# Autodesk Inventor assembly: ASY MSC 002 отстойник осветлитель
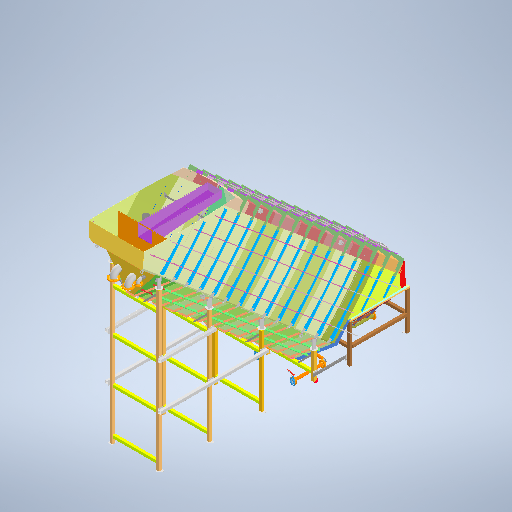
[picture p0: Inventor's stored thumbnail of the model, 512x512]
Saved by Autodesk Inventor 2025 (Build 290162010, 162A)
## iProperties
allow_slope_adjustment: 0 ul
flow_configuration: 1 ul
flow_direction: 2 ul
loss_method: 0 ul
radius: 110.000 mm
flow_configuration2: 1 ul
radius: 61.000 mm
radius: 44.450 mm
radius: 59.000 mm
Created: 2024-09-05
Part Number: ASY MSC 002 отстойник осветлитель
Document SubType Name: Assembly
Designer: admin
Mass: 3.32015e+06 g
Surface Area: 6.08051e+06 cm^2
Volume: 432456 cm^3
Author: admin
## Documents named in this file (64)
- C:\Users\pokla\Documents\Inventor\Отстойник осветлитель\Manturovo_Se-clar-Gleb\ASY MSC 002 отстойник осветлитель.iam
- C:\Users\pokla\Documents\Inventor\Отстойник осветлитель\Manturovo_Se-clar-Gleb\ASY MSC 900.1 base frame.iam
- C:\Users\pokla\Documents\Inventor\Отстойник осветлитель\Manturovo_Se-clar-Gleb\ASY MSC 100 cone.iam
- C:\Users\pokla\Documents\Inventor\Отстойник осветлитель\Manturovo_Se-clar-Gleb\MSC 401 sheet lowerback.ipt
- C:\Users\pokla\Documents\Inventor\Отстойник осветлитель\Manturovo_Se-clar-Gleb\MSC 701 face 1.ipt
- C:\Users\pokla\Documents\Inventor\Отстойник осветлитель\Manturovo_Se-clar-Gleb\MSC 705 ridge 3.ipt
- C:\Users\pokla\Documents\Inventor\Отстойник осветлитель\Manturovo_Se-clar-Gleb\MSC 713 tube.ipt
- C:\Users\pokla\Documents\Inventor\Отстойник осветлитель\Manturovo_Se-clar-Gleb\ISO 5251 Bends 3D without straight ends(90 deg) DN150 11 11.ipt
- C:\Users\pokla\Documents\Inventor\Отстойник осветлитель\Manturovo_Se-clar-Gleb\MSC 408 stringer lowerback.ipt
- C:\Users\pokla\Documents\Inventor\Отстойник осветлитель\Manturovo_Se-clar-Gleb\MSC 703 face 2.ipt
- C:\Users\pokla\Documents\Inventor\Отстойник осветлитель\Manturovo_Se-clar-Gleb\MSC 702 face 3.ipt
- C:\Users\pokla\Documents\Inventor\Отстойник осветлитель\Manturovo_Se-clar-Gleb\MSC 704 face 4.ipt
- C:\Users\pokla\Documents\Inventor\Отстойник осветлитель\Manturovo_Se-clar-Gleb\ASY MSC 900.3 base frame.iam
- C:\Users\pokla\Documents\Inventor\Отстойник осветлитель\Manturovo_Se-clar-Gleb\Pillars\ASY MSC 900.5 base frame.iam
- C:\Users\pokla\Documents\Inventor\Отстойник осветлитель\Manturovo_Se-clar-Gleb\Pillars\ASY MSC 900.4  base frame.iam
- C:\Users\pokla\Documents\Inventor\Отстойник осветлитель\Manturovo_Se-clar-Gleb\Pillars\ASY MSC 900.6 base frame.iam
- C:\Users\pokla\Documents\Inventor\Отстойник осветлитель\Manturovo_Se-clar-Gleb\ASY MSC 200 BACK.iam
- C:\Users\pokla\Documents\Inventor\Отстойник осветлитель\Manturovo_Se-clar-Gleb\ASY MSC 300.2 LEFT BOARD.iam
- C:\Users\pokla\Documents\Inventor\Отстойник осветлитель\Manturovo_Se-clar-Gleb\ASY MSC 300.1 RIGHT BOARD.iam
- C:\Users\pokla\Documents\Inventor\Отстойник осветлитель\Manturovo_Se-clar-Gleb\ASY MSC 500 BELLY.iam
- C:\Users\pokla\Documents\Inventor\Отстойник осветлитель\Manturovo_Se-clar-Gleb\ASY MSC 900.2 support.iam
- C:\Users\pokla\Documents\Inventor\Отстойник осветлитель\Manturovo_Se-clar-Gleb\ASY MSC 600 cone exit back.iam
- C:\Users\pokla\Documents\Inventor\Отстойник осветлитель\Manturovo_Se-clar-Gleb\ASY MSC 800 gills.iam
- C:\Users\pokla\Documents\Inventor\Отстойник осветлитель\Manturovo_Se-clar-Gleb\ASY MSC 400 Accsess hatch.iam
- C:\Users\pokla\Documents\Inventor\Отстойник осветлитель\Manturovo_Se-clar-Gleb\MSC DIM 000 settler-clarifier.ipt
- C:\Users\pokla\Documents\Inventor\Отстойник осветлитель\Manturovo_Se-clar-Gleb\MSC DIM 001 frame.ipt
- C:\Users\pokla\Documents\Inventor\Отстойник осветлитель\Manturovo_Se-clar-Gleb\ASY MSC 900.7 base frame transverse.iam
- C:\Users\pokla\Documents\Inventor\Отстойник осветлитель\Manturovo_Se-clar-Gleb\ASY MSC 900.8 base frame transverse.iam
- C:\Users\pokla\Documents\Inventor\Отстойник осветлитель\Manturovo_Se-clar-Gleb\MSC 908 transverse pillar plate.ipt
- C:\Users\pokla\Documents\Inventor\Отстойник осветлитель\Manturovo_Se-clar-Gleb\MSC 900.9 base frame transverse.ipt
- C:\Users\pokla\Documents\Inventor\Отстойник осветлитель\Manturovo_Se-clar-Gleb\ASY MSC 700 water tray.iam
- C:\Users\pokla\Documents\Inventor\Отстойник осветлитель\Manturovo_Se-clar-Gleb\ASY 940 linkage.iam
- C:\Users\pokla\Documents\Inventor\Отстойник осветлитель\Manturovo_Se-clar-Gleb\MSC 510 BELLY PILLAR.ipt
- C:\Users\pokla\Documents\Inventor\Отстойник осветлитель\Manturovo_Se-clar-Gleb\ASY MSC 900.7 support.iam
- C:\Users\pokla\Documents\Inventor\Отстойник осветлитель\Manturovo_Se-clar-Gleb\Content Center Files\en-US\DIN 2605 90 T 3\DIN 2605 90 Deg Elbow Type 2 168.3 - 2.6S.ipt
- C:\Users\admin\YandexDisk-badmisterfox\домашниий пк\Inventor\Manturovo\Manturovo_Se-clar\3d party\Stamp flange DIN2642\Stamd flange lapped collar DIN2642.ipt
- C:\Users\pokla\Documents\Inventor\Отстойник осветлитель\Manturovo_Se-clar-Gleb\3d party\Stamp flange DIN2642\Stamd flange lapped collar DIN2642\Stamp flange DIN2642-150.ipt
- C:\Users\pokla\Documents\Inventor\Отстойник осветлитель\Manturovo_Se-clar-Gleb\Content Center Files\en-US\DIN 2605 90 T 3\DIN 2605 90 Deg Elbow Type 2 88.9 - 2.3S.ipt
- C:\Users\pokla\Documents\Inventor\Отстойник осветлитель\Manturovo_Se-clar-Gleb\Stamp flange DIN2642-080.ipt
- C:\Users\pokla\Documents\Inventor\Отстойник осветлитель\Manturovo_Se-clar-Gleb\DIN EN ISO 1127(1) - 88,9 x 2,3 - 100.ipt
- C:\Users\pokla\Documents\Inventor\Отстойник осветлитель\Manturovo_Se-clar-Gleb\3d party\Butterfly value\butterfly-valve-3-in-1.snapshot.4\vpe_3449-02_dn80_.iam
- C:\Users\pokla\Documents\Inventor\Отстойник осветлитель\Manturovo_Se-clar-Gleb\MSC 606 rocket tube 6.ipt
- C:\Users\pokla\Documents\Inventor\Отстойник осветлитель\Manturovo_Se-clar-Gleb\Stamp flange DIN2642-065.ipt
- C:\Users\pokla\Documents\Inventor\Отстойник осветлитель\Manturovo_Se-clar-Gleb\ContentCenter\en-US\ISO 5251 B 3D\ISO 5251 Bends 3D without straight ends(90 deg) DN65 2.9 2.9.ipt
- C:\Users\pokla\Documents\Inventor\Отстойник осветлитель\Manturovo_Se-clar-Gleb\MSC 616 belly tube 16.ipt
- C:\Users\pokla\Documents\Inventor\Отстойник осветлитель\Manturovo_Se-clar-Gleb\MSC 617 belly tube 17.ipt
- C:\Users\pokla\Documents\Inventor\Отстойник осветлитель\Manturovo_Se-clar-Gleb\MSC 618 belly tube 18.ipt
- C:\Users\pokla\Documents\Inventor\Отстойник осветлитель\Manturovo_Se-clar-Gleb\MSC 808 sheet.ipt
- C:\Users\pokla\Documents\Inventor\Отстойник осветлитель\Manturovo_Se-clar-Gleb\DIN EN 10219-2 - 40 x 20 x 2  - 2000.ipt
- C:\Users\pokla\Documents\Inventor\Отстойник осветлитель\Manturovo_Se-clar-Gleb\ISO 4019 - 40x20x2 - 1600.ipt
- C:\Users\pokla\Documents\Inventor\Отстойник осветлитель\Manturovo_Se-clar-Gleb\MSC 814 wall inner rib.ipt
- C:\Users\pokla\Documents\Inventor\Отстойник осветлитель\Manturovo_Se-clar-Gleb\MSC 815 wall inner.ipt
- C:\Users\pokla\Documents\Inventor\Отстойник осветлитель\Manturovo_Se-clar-Gleb\MSC 815 wall inner joint.ipt
- C:\Users\pokla\Documents\Inventor\Отстойник осветлитель\Manturovo_Se-clar-Gleb\UNI EN ISO 1127(1) - 168.3 x 2 - 700.ipt
- C:\Users\pokla\Documents\Inventor\Отстойник осветлитель\Manturovo_Se-clar-Gleb\MSC 912 flange slipway.ipt
- C:\Users\pokla\Documents\Inventor\Отстойник осветлитель\Manturovo_Se-clar-Gleb\MSC 913 flange slipway.ipt
- C:\Users\pokla\Documents\Inventor\Отстойник осветлитель\Manturovo_Se-clar-Gleb\MSC 920 plug 88.9.ipt
- C:\Users\pokla\Documents\Inventor\Отстойник осветлитель\Manturovo_Se-clar-Gleb\MSC 921 plug 76.ipt
- C:\Users\pokla\Documents\Inventor\Отстойник осветлитель\Manturovo_Se-clar-Gleb\MSC 922 plug 76 hole.ipt
- C:\Users\pokla\Documents\Inventor\Отстойник осветлитель\Manturovo_Se-clar-Gleb\MSC 922 plug 150.ipt
- C:\Users\pokla\Documents\Inventor\Отстойник осветлитель\Manturovo_Se-clar-Gleb\AQUA AISI304 4vv wheel plate 150.ipt
- C:\Users\pokla\Documents\Inventor\Отстойник осветлитель\Manturovo_Se-clar-Gleb\MSC 923 step .ipt
- C:\Users\pokla\Documents\Inventor\Отстойник осветлитель\Manturovo_Se-clar-Gleb\ASY MSC D-ring.iam
- C:\Users\pokla\Documents\Inventor\Отстойник осветлитель\Manturovo_Se-clar-Gleb\3d party\Stamp flange DIN2642\Stamd flange lapped collar DIN2642.ipt
## Components (104 placed, 62 different names)
1. MSC DIM 000 settler-clarifier.ipt:1
2. MSC DIM 001 frame.ipt:1
3. ASY MSC 900.4  base frame.iam:1 [sub-assembly] — Mate:32, Mate:33, Mate:45, Mate:46, Cylindrical:11, Mate:82, Rigid:67
4. ASY MSC 900.5 base frame.iam:1 [sub-assembly] — Flush:11, Cylindrical:7, Mate:46, Mate:48, Cylindrical:10
5. ASY MSC 900.6 base frame.iam:1 [sub-assembly] — Mate:38, Mate:39, Cylindrical:6, Mate:47, Rigid:19, Rigid:20, Rigid:21, Rigid:22, Cylindrical:9, Mate:84
6. ASY MSC 900.3 base frame.iam:1 [sub-assembly] — Mate:23, Mate:24, Mate:44, Mate:45, Rigid:31, Rigid:32, Rigid:33, Cylindrical:8
7. ASY MSC 900.8 base frame transverse.iam:1 [sub-assembly] — Rigid:22
8. ASY MSC 900.8 base frame transverse.iam:2 [sub-assembly] — Rigid:21
9. ASY MSC 900.7 base frame transverse.iam:1 [sub-assembly] — Rigid:19
10. ASY MSC 900.7 base frame transverse.iam:2 [sub-assembly] — Rigid:20
11. ASY MSC 900.2 support.iam:5 [sub-assembly]
12. ASY MSC 900.7 support:2 [sub-assembly] — Cylindrical:11, Mate:78
13. ASY MSC 900.2 support.iam:4 [sub-assembly] — Cylindrical:7, Mate:41
14. ASY MSC 900.7 support:3 [sub-assembly] — Cylindrical:10, Mate:79
15. ASY MSC 900.2 support.iam:1 [sub-assembly] — Cylindrical:6, Mate:42
16. ASY MSC 900.7 support:4 [sub-assembly] — Cylindrical:9, Mate:80
17. ASY MSC 900.2 support.iam:8 [sub-assembly]
18. ASY MSC 900.7 support:1 [sub-assembly] — Cylindrical:8, Mate:77
19. ASY MSC 600 cone exit back.iam:1 [sub-assembly] — Rigid:17, Mate:94, Flush:34
20. ASY MSC 700 water tray.iam:1 [sub-assembly] — Flush:22, Tangent:1
21. ASY MSC 400 Accsess hatch.iam:1 [sub-assembly] — Mate:99, Cylindrical:12
22. ASY MSC 100 cone.iam:1 [sub-assembly] — Mate:19, Flush:6, Rigid:17, Rigid:53, Rigid:69, Rigid:71, Rigid:72, Flush:35
23. MSC 401 sheet lowerback.ipt:1 — Cylindrical:12, Flush:35, Flush:36
24. MSC 705 ridge 3.ipt:1 — Flush:19, Flush:20
25. MSC 704 face 4.ipt:1 — Mate:89, Mate:100
26. MSC 900.9 base frame transverse.ipt:4 — Mate:81, Mate:83
27. Part1:2 — Mate:81, Mate:82
28. Part1:4 — Mate:88
29. MSC 900.9 base frame transverse:7 — Mate:87, Mate:88
30. Part1:3 — Mate:84, Mate:85
31. MSC 900.9 base frame transverse.ipt:1 — Mate:85, Mate:86
32. MSC 701 face 1.ipt:1 — Rigid:4, Flush:9, Mate:35, Rigid:35, Rigid:36, Rigid:39, Rigid:40, Mate:100
33. MSC 702 face 3.ipt:1 — Mate:34, Mate:35, Mate:36, Mate:66, Mate:102, Mate:103
34. MSC 703 face 2.ipt:1 — Flush:13, Flush:17, Mate:66, Flush:19
35. ISO 5251 Bends 3D without straight ends(90 deg) DN150 11 11.ipt:1 — Rigid:66
36. MSC 713 tube.ipt:1 — Rigid:4
37. Part1.ipt:1 — Rigid:33, Mate:68, Mate:69, Mate:70
38. MSC 900.9 base frame transverse.ipt:3 — Mate:68, Mate:69, Mate:70
39. MSC 908 transverse pillar plate.ipt:1
40. MSC 908 transverse pillar plate.ipt:2 — Mate:50, Flush:16, Flush:18
41. MSC 408 stringer lowerback.ipt:2
42. MSC 408 stringer lowerback.ipt:1
43. ASY MSC 900.1 base frame.iam:1 [sub-assembly] — Flush:5, Mate:19, Mate:44, Mate:47, Mate:50, Flush:16, Rigid:68
44. ASY 940 linkage.iam:1 [sub-assembly] — Rigid:32, Flush:18
45. ASY 940 linkage.iam:2 [sub-assembly] — Rigid:31
46. ASY MSC 500 BELLY.iam:1 [sub-assembly] — Flush:7, Mate:22, Rigid:10, Rigid:11, Mate:41, Mate:42, Mate:77, Mate:78, Mate:79, Mate:80, Mate:83, Mate:86, Mate:87
47. ASY MSC 200 BACK.iam:1 [sub-assembly] — Flush:8
48. ASY MSC 300.2 LEFT BOARD.iam:1 [sub-assembly] — Rigid:11, Mate:34
49. ASY MSC 300.1 RIGHT BOARD.iam:1 [sub-assembly] — Rigid:10, Flush:17
50. ASY MSC 800 gills.iam:1 [sub-assembly] — Mate:22, Mate:94, Rigid:56, Rigid:57, Mate:111
51. DIN 2605 90 Deg Elbow Type 2 168.3 - 2.6S:1 — Rigid:36, Rigid:38
52. DIN 2605 90 Deg Elbow Type 2 168.3 - 2.6S:2 — Rigid:35, Rigid:37
53. Stamp flange DIN2642-150:1 — Rigid:38, Rotational:9
54. Stamp flange DIN2642-150:3 — Rigid:37, Rigid:73
55. DIN 2605 90 Deg Elbow Type 2 88.9 - 2.3S:1 — Rigid:39, Rotational:2
56. Stamp flange DIN2642-080:4 — Rotational:2, Rigid:70
57. DIN EN ISO 1127(1) - 88,9 x 2,3 - 100:1 — Rigid:40
58. MSC 606 rocket tube 6.ipt:1 — Rotational:4
59. ISO 5251 Bends 3D without straight ends(90 deg) DN65 2.9:1 — Rigid:45, Rigid:47
60. Stamp flange DIN2642-065.ipt:1 — Rotational:3, Rotational:6
61. ISO 5251 Bends 3D without straight ends(90 deg) DN65 2.9:2 — Rotational:3, Rigid:46
62. MSC 616 belly tube 16:1 — Rigid:45, Rigid:46
63. Stamp flange DIN2642-065:6 — Rigid:47, Rotational:5
64. Stamp flange DIN2642-065:7 — Rotational:4, Rotational:5, Rotational:8
65. Stamp flange DIN2642-065:8 — Rotational:6, Rotational:7
66. MSC 617 belly tube 17:1 — Rotational:7, Rigid:50
67. Stamp flange DIN2642-065:9 — Rigid:50, Rigid:55
68. MSC 618 belly tube 18:1 — Rigid:52, Rigid:51
69. Stamp flange DIN2642-065:10 — Rigid:53, Rigid:52
70. Stamp flange DIN2642-065:11 — Rigid:51, Rigid:54
71. vpe_3449-02_dn80_:2 [sub-assembly] — Rigid:54
72. vpe_3449-02_dn80_:3 [sub-assembly] — Rigid:55
73. MSC 808 sheet:1
74. DIN EN 10219-2 - 40 x 20 x 2  - 2000:1
75. ISO 4019 - 40x20x2 - 1600:1 — Mate:95, Rigid:63, Rigid:64, Flush:22, Tangent:1
76. ISO 4019 - 40x20x2 - 1600:2 — Mate:92, Mate:97
77. MSC 814 wall inner rib:1 — Rigid:56, Mate:97, Rigid:59, Rigid:61
78. MSC 814 wall inner rib:2 — Rigid:57, Rigid:58, Rigid:60, Rigid:74
79. MSC 815 wall inner:1 — Rigid:58
80. MSC 815 wall inner:2 — Rigid:59
81. MSC 815 wall inner:3 — Rigid:60, Rigid:76
82. MSC 815 wall inner:4 — Rigid:61
83. MSC 815 wall inner joint:1 — Rigid:62
84. MSC 815 wall inner:5 — Rigid:63, Rigid:62
85. MSC 815 wall inner:6 — Rigid:64, Rigid:65
86. MSC 815 wall inner joint:2 — Rigid:65
87. UNI EN ISO 1127(1) - 168.3 x 2 - 700:1 — Rigid:66
88. MSC 912 flange slipway:1 — Rigid:67
89. MSC 913 flange slipway:1 — Rigid:68
90. Part1:5 — Rigid:69
91. MSC 921 plug 76:1 — Rotational:8
92. Part1:6 — Rigid:70
93. MSC 922 plug 76 hole:1 — Rigid:71
94. vpe_3449-02_dn80_:4 [sub-assembly] — Rigid:72
95. MSC 922 plug 150:1 — Rigid:73
96. MSC 922 plug 150:2 — Rotational:9
97. Part1:7 — Flush:32
98. MSC 923 step :1
99. ASY MSC D-ring:2 [sub-assembly] — Mate:102, Flush:33
100. ASY MSC D-ring:3 [sub-assembly] — Mate:103, Flush:33
101. MSC 815 wall inner:7 — Rigid:74, Rigid:75
102. ISO 4019 - 40x20x2 - 1600:3 — Rigid:75
103. ISO 4019 - 40x20x2 - 1600:4 — Rigid:76
104. MSC 815 wall inner:8 — Mate:111
## Relationships (144: Mate 54, WeldJoint 53, Flush 19, CylindricalJoint 9, RevoluteJoint 8, Tangent 1)
- [WeldJoint]: ISO 5251 Bends 3D without straight ends(90 deg) DN150 11 11.ipt:1 ↔ MSC 713 tube.ipt:1
- [Mate]: ASY MSC 100 cone.iam:1 ↔ MSC 408 stringer lowerback.ipt:1
- Rigid:4 [WeldJoint]: MSC 701 face 1.ipt:1 ↔ MSC 713 tube.ipt:1
- [Mate]: ASY MSC 100 cone.iam:1 ↔ MSC 408 stringer lowerback.ipt:2
- [Mate]: ASY MSC 600 cone exit back.iam:1 ↔ ASY MSC 500 BELLY.iam:1
- [WeldJoint]: ASY MSC 700 water tray.iam:1 ↔ MSC 705 ridge 3.ipt:1
- [WeldJoint]: ASY MSC 700 water tray.iam:1 ↔ MSC 705 ridge 3.ipt:1
- [Mate]: ASY MSC 500 BELLY.iam:1 ↔ ASY MSC 800 gills.iam:1
- [Mate]: MSC 701 face 1.ipt:1 ↔ ASY MSC 500 BELLY.iam:1
- [Mate] (3 mm): MSC 701 face 1.ipt:1 ↔ ASY MSC 500 BELLY.iam:1
- [Mate] (3 mm): ASY MSC 900.2 support.iam:5 ↔ ASY MSC 500 BELLY.iam:1
- [Mate] (3 mm): ASY MSC 900.2 support.iam:8 ↔ ASY MSC 500 BELLY.iam:1
- [CylindricalJoint]: ASY MSC 900.4  base frame.iam:1 ↔ ASY MSC 900.2 support.iam:5
- [Mate] (-2860 mm): ASY MSC 500 BELLY.iam:1 ↔ ASY MSC 200 BACK.iam:1
- [CylindricalJoint]: ASY MSC 900.3 base frame.iam:1 ↔ ASY MSC 900.2 support.iam:8
- [Flush]: ASY MSC 900.4  base frame.iam:1 ↔ ASY MSC 900.3 base frame.iam:1
- Flush:5: ASY MSC 900.1 base frame.iam:1
- Mate:19: ASY MSC 100 cone.iam:1 ↔ ASY MSC 900.1 base frame.iam:1
- Flush:6: ASY MSC 100 cone.iam:1
- Flush:7: ASY MSC 500 BELLY.iam:1
- Flush:8: ASY MSC 200 BACK.iam:1
- Mate:22: ASY MSC 500 BELLY.iam:1 ↔ ASY MSC 800 gills.iam:1
- Mate:23: ASY MSC 900.3 base frame.iam:1
- Mate:24: ASY MSC 900.3 base frame.iam:1
- Flush:9: MSC 701 face 1.ipt:1
- Rigid:10 [WeldJoint] (-25 mm): ASY MSC 500 BELLY.iam:1 ↔ ASY MSC 300.1 RIGHT BOARD.iam:1
- Rigid:11 [WeldJoint] (-25 mm): ASY MSC 500 BELLY.iam:1 ↔ ASY MSC 300.2 LEFT BOARD.iam:1
- Flush:11: ASY MSC 900.5 base frame.iam:1
- Mate:32: ASY MSC 900.4  base frame.iam:1
- Mate:33: ASY MSC 900.4  base frame.iam:1
- Mate:34: MSC 702 face 3.ipt:1 ↔ ASY MSC 300.2 LEFT BOARD.iam:1
- Mate:35: MSC 701 face 1.ipt:1 ↔ MSC 702 face 3.ipt:1
- [WeldJoint]: ASY MSC 700 water tray.iam:1 ↔ MSC 705 ridge 3.ipt:1
- Mate:36: MSC 702 face 3.ipt:1
- Mate:38: ASY MSC 900.6 base frame.iam:1
- Mate:39: ASY MSC 900.6 base frame.iam:1
- Cylindrical:6: ASY MSC 900.6 base frame.iam:1 ↔ ASY MSC 900.2 support.iam:1
- Cylindrical:7: ASY MSC 900.5 base frame.iam:1 ↔ ASY MSC 900.2 support.iam:4
- Mate:41 (3 mm): ASY MSC 900.2 support.iam:4 ↔ ASY MSC 500 BELLY.iam:1
- Mate:42 (3 mm): ASY MSC 900.2 support.iam:1 ↔ ASY MSC 500 BELLY.iam:1
- Flush:13: MSC 703 face 2.ipt:1
- Mate:44 (820 mm): ASY MSC 900.3 base frame.iam:1 ↔ ASY MSC 900.1 base frame.iam:1
- Mate:45 (1430 mm): ASY MSC 900.4  base frame.iam:1 ↔ ASY MSC 900.3 base frame.iam:1
- Mate:46 (1430 mm): ASY MSC 900.4  base frame.iam:1 ↔ ASY MSC 900.5 base frame.iam:1
- Mate:47 (5300 mm): ASY MSC 900.6 base frame.iam:1 ↔ ASY MSC 900.1 base frame.iam:1
- Rigid:17 [WeldJoint]: ASY MSC 600 cone exit back.iam:1 ↔ ASY MSC 100 cone.iam:1
- Mate:48: ASY MSC 900.5 base frame.iam:1
- Rigid:19 [WeldJoint]: ASY MSC 900.6 base frame.iam:1 ↔ ASY MSC 900.7 base frame transverse.iam:1
- Rigid:20 [WeldJoint]: ASY MSC 900.6 base frame.iam:1 ↔ ASY MSC 900.7 base frame transverse.iam:2
- Rigid:21 [WeldJoint]: ASY MSC 900.6 base frame.iam:1 ↔ ASY MSC 900.8 base frame transverse.iam:2
- Rigid:22 [WeldJoint]: ASY MSC 900.6 base frame.iam:1 ↔ ASY MSC 900.8 base frame transverse.iam:1
- Mate:50: MSC 908 transverse pillar plate.ipt:2 ↔ ASY MSC 900.1 base frame.iam:1
- Flush:16 (-40 mm): MSC 908 transverse pillar plate.ipt:2 ↔ ASY MSC 900.1 base frame.iam:1
- Flush:17: MSC 703 face 2.ipt:1 ↔ ASY MSC 300.1 RIGHT BOARD.iam:1
- Mate:66: MSC 702 face 3.ipt:1 ↔ MSC 703 face 2.ipt:1
- [WeldJoint]: MSC 908 transverse pillar plate.ipt:1 ↔ ASY 940 linkage.iam:2
- Rigid:31 [WeldJoint]: ASY MSC 900.3 base frame.iam:1 ↔ ASY 940 linkage.iam:2
- Rigid:32 [WeldJoint]: ASY MSC 900.3 base frame.iam:1 ↔ ASY 940 linkage.iam:1
- Flush:18: MSC 908 transverse pillar plate.ipt:2 ↔ ASY 940 linkage.iam:1
- Rigid:33 [WeldJoint]: ASY MSC 900.3 base frame.iam:1 ↔ Part1.ipt:1
- Mate:68: Part1.ipt:1 ↔ MSC 900.9 base frame transverse.ipt:3
- Mate:69 (11 mm): Part1.ipt:1 ↔ MSC 900.9 base frame transverse.ipt:3
- Mate:70: Part1.ipt:1 ↔ MSC 900.9 base frame transverse.ipt:3
- Cylindrical:8: ASY MSC 900.3 base frame.iam:1 ↔ ASY MSC 900.7 support:1
- Mate:77: ASY MSC 900.7 support:1 ↔ ASY MSC 500 BELLY.iam:1
- Cylindrical:9: ASY MSC 900.6 base frame.iam:1 ↔ ASY MSC 900.7 support:4
- Cylindrical:10: ASY MSC 900.5 base frame.iam:1 ↔ ASY MSC 900.7 support:3
- Cylindrical:11: ASY MSC 900.4  base frame.iam:1 ↔ ASY MSC 900.7 support:2
- Mate:78: ASY MSC 900.7 support:2 ↔ ASY MSC 500 BELLY.iam:1
- Mate:79: ASY MSC 900.7 support:3 ↔ ASY MSC 500 BELLY.iam:1
- Mate:80: ASY MSC 900.7 support:4 ↔ ASY MSC 500 BELLY.iam:1
- Mate:81: MSC 900.9 base frame transverse.ipt:4 ↔ Part1:2
- Mate:82: ASY MSC 900.4  base frame.iam:1 ↔ Part1:2
- Mate:83: MSC 900.9 base frame transverse.ipt:4 ↔ ASY MSC 500 BELLY.iam:1
- Mate:84: ASY MSC 900.6 base frame.iam:1 ↔ Part1:3
- Mate:85: Part1:3 ↔ MSC 900.9 base frame transverse.ipt:1
- Mate:86: MSC 900.9 base frame transverse.ipt:1 ↔ ASY MSC 500 BELLY.iam:1
- Mate:87: MSC 900.9 base frame transverse:7 ↔ ASY MSC 500 BELLY.iam:1
- Mate:88: Part1:4 ↔ MSC 900.9 base frame transverse:7
- Rigid:35 [WeldJoint]: MSC 701 face 1.ipt:1 ↔ DIN 2605 90 Deg Elbow Type 2 168.3 - 2.6S:2
- Rigid:36 [WeldJoint]: MSC 701 face 1.ipt:1 ↔ DIN 2605 90 Deg Elbow Type 2 168.3 - 2.6S:1
- Rigid:37 [WeldJoint]: DIN 2605 90 Deg Elbow Type 2 168.3 - 2.6S:2 ↔ Stamp flange DIN2642-150:3
- Rigid:38 [WeldJoint]: DIN 2605 90 Deg Elbow Type 2 168.3 - 2.6S:1 ↔ Stamp flange DIN2642-150:1
- Rigid:39 [WeldJoint] (-100 mm): MSC 701 face 1.ipt:1 ↔ DIN 2605 90 Deg Elbow Type 2 88.9 - 2.3S:1
- Rotational:2 [RevoluteJoint]: DIN 2605 90 Deg Elbow Type 2 88.9 - 2.3S:1 ↔ Stamp flange DIN2642-080:4
- Rigid:40 [WeldJoint]: MSC 701 face 1.ipt:1 ↔ DIN EN ISO 1127(1) - 88,9 x 2,3 - 100:1
- [WeldJoint]: ASY MSC 600 cone exit back.iam:1 ↔ MSC 606 rocket tube 6.ipt:1
- Rotational:3 [RevoluteJoint]: Stamp flange DIN2642-065.ipt:1 ↔ ISO 5251 Bends 3D without straight ends(90 deg) DN65 2.9:2
- Rigid:45 [WeldJoint]: ISO 5251 Bends 3D without straight ends(90 deg) DN65 2.9:1 ↔ MSC 616 belly tube 16:1
- Rigid:46 [WeldJoint]: ISO 5251 Bends 3D without straight ends(90 deg) DN65 2.9:2 ↔ MSC 616 belly tube 16:1
- Rigid:47 [WeldJoint]: ISO 5251 Bends 3D without straight ends(90 deg) DN65 2.9:1 ↔ Stamp flange DIN2642-065:6
- Rotational:4 [RevoluteJoint]: MSC 606 rocket tube 6.ipt:1 ↔ Stamp flange DIN2642-065:7
- Rotational:5 [RevoluteJoint]: Stamp flange DIN2642-065:6 ↔ Stamp flange DIN2642-065:7
- Rotational:6 [RevoluteJoint]: Stamp flange DIN2642-065.ipt:1 ↔ Stamp flange DIN2642-065:8
- Rotational:7 [RevoluteJoint]: Stamp flange DIN2642-065:8 ↔ MSC 617 belly tube 17:1
- Rigid:50 [WeldJoint]: MSC 617 belly tube 17:1 ↔ Stamp flange DIN2642-065:9
- Rigid:53 [WeldJoint]: ASY MSC 100 cone.iam:1 ↔ Stamp flange DIN2642-065:10
- Rigid:52 [WeldJoint]: MSC 618 belly tube 18:1 ↔ Stamp flange DIN2642-065:10
- Rigid:51 [WeldJoint]: MSC 618 belly tube 18:1 ↔ Stamp flange DIN2642-065:11
- Rigid:54 [WeldJoint]: Stamp flange DIN2642-065:11 ↔ vpe_3449-02_dn80_:2
- Rigid:55 [WeldJoint]: Stamp flange DIN2642-065:9 ↔ vpe_3449-02_dn80_:3
- Flush:19 (170 mm): MSC 705 ridge 3.ipt:1 ↔ MSC 703 face 2.ipt:1
- Flush:20: MSC 705 ridge 3.ipt:1
- Mate:89: MSC 704 face 4.ipt:1
- Mate:92: ISO 4019 - 40x20x2 - 1600:2
- Mate:94 (1100 mm): ASY MSC 600 cone exit back.iam:1 ↔ ASY MSC 800 gills.iam:1
- Mate:95: ISO 4019 - 40x20x2 - 1600:1
- Rigid:56 [WeldJoint] (650 mm): ASY MSC 800 gills.iam:1 ↔ MSC 814 wall inner rib:1
- Rigid:57 [WeldJoint] (650 mm): ASY MSC 800 gills.iam:1 ↔ MSC 814 wall inner rib:2
- Mate:97 (3 mm): ISO 4019 - 40x20x2 - 1600:2 ↔ MSC 814 wall inner rib:1
- Rigid:58 [WeldJoint]: MSC 814 wall inner rib:2 ↔ MSC 815 wall inner:1
- Rigid:59 [WeldJoint]: MSC 814 wall inner rib:1 ↔ MSC 815 wall inner:2
- Rigid:60 [WeldJoint]: MSC 814 wall inner rib:2 ↔ MSC 815 wall inner:3
- Rigid:61 [WeldJoint]: MSC 814 wall inner rib:1 ↔ MSC 815 wall inner:4
- Rigid:62 [WeldJoint]: MSC 815 wall inner joint:1 ↔ MSC 815 wall inner:5
- Rigid:63 [WeldJoint] (8 mm): ISO 4019 - 40x20x2 - 1600:1 ↔ MSC 815 wall inner:5
- Rigid:64 [WeldJoint] (8 mm): ISO 4019 - 40x20x2 - 1600:1 ↔ MSC 815 wall inner:6
- Flush:22 (666 mm): ASY MSC 700 water tray.iam:1 ↔ ISO 4019 - 40x20x2 - 1600:1
- Tangent:1: ASY MSC 700 water tray.iam:1 ↔ ISO 4019 - 40x20x2 - 1600:1
- Rigid:65 [WeldJoint]: MSC 815 wall inner:6 ↔ MSC 815 wall inner joint:2
- Mate:99: ASY MSC 400 Accsess hatch.iam:1
- Cylindrical:12: ASY MSC 400 Accsess hatch.iam:1 ↔ MSC 401 sheet lowerback.ipt:1
- Rigid:66 [WeldJoint]: ISO 5251 Bends 3D without straight ends(90 deg) DN150 11 11.ipt:1 ↔ UNI EN ISO 1127(1) - 168.3 x 2 - 700:1
- Rigid:67 [WeldJoint]: ASY MSC 900.4  base frame.iam:1 ↔ MSC 912 flange slipway:1
- Mate:100: MSC 704 face 4.ipt:1 ↔ MSC 701 face 1.ipt:1
- Rigid:68 [WeldJoint]: ASY MSC 900.1 base frame.iam:1 ↔ MSC 913 flange slipway:1
- Rigid:69 [WeldJoint]: ASY MSC 100 cone.iam:1 ↔ Part1:5
- Rotational:8 [RevoluteJoint]: Stamp flange DIN2642-065:7 ↔ MSC 921 plug 76:1
- Rigid:70 [WeldJoint]: Stamp flange DIN2642-080:4 ↔ Part1:6
- Rigid:71 [WeldJoint] (49 mm): ASY MSC 100 cone.iam:1 ↔ MSC 922 plug 76 hole:1
- Rigid:72 [WeldJoint]: ASY MSC 100 cone.iam:1 ↔ vpe_3449-02_dn80_:4
- Rigid:73 [WeldJoint]: Stamp flange DIN2642-150:3 ↔ MSC 922 plug 150:1
- Rotational:9 [RevoluteJoint]: Stamp flange DIN2642-150:1 ↔ MSC 922 plug 150:2
- Flush:32: Part1:7
- Mate:102: MSC 702 face 3.ipt:1 ↔ ASY MSC D-ring:2
- Mate:103: MSC 702 face 3.ipt:1 ↔ ASY MSC D-ring:3
- Flush:33: ASY MSC D-ring:2 ↔ ASY MSC D-ring:3
- Rigid:74 [WeldJoint]: MSC 814 wall inner rib:2 ↔ MSC 815 wall inner:7
- Rigid:75 [WeldJoint]: MSC 815 wall inner:7 ↔ ISO 4019 - 40x20x2 - 1600:3
- Rigid:76 [WeldJoint]: MSC 815 wall inner:3 ↔ ISO 4019 - 40x20x2 - 1600:4
- Mate:111: ASY MSC 800 gills.iam:1 ↔ MSC 815 wall inner:8
- Flush:34: ASY MSC 600 cone exit back.iam:1
- Flush:35: ASY MSC 100 cone.iam:1 ↔ MSC 401 sheet lowerback.ipt:1
- Flush:36: MSC 401 sheet lowerback.ipt:1
## Named parameters: d334_d122 = 0 mm
